# Autodesk Inventor assembly: Intake Assembly
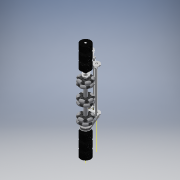
[picture p0: Inventor's stored thumbnail of the model, 180x180]
Saved by Autodesk Inventor 2019.4 (Build 234330000, 330)
## iProperties
Created: 2020-01-28
Part Number: Intake Assembly
Document SubType Name: Assembly
Designer: admin
Mass: 2236.14 g
Surface Area: 6786.27 cm^2
Volume: 1184.94 cm^3
Density: 1.88713 g/cm^3
Author: admin
## Documents named in this file (15)
- C:\Users\admin\Desktop\FRC 2020 Engineering\GitHub\7738-2020\Robot V2\Intake V2\Intake Assembly.iam
- C:\Users\admin\Desktop\FRC 2020 Engineering\GitHub\7738-2020\Robot V2\Intake V2\Intake Arm.ipt
- C:\Users\admin\Desktop\FRC 2020 Engineering\GitHub\7738-2020\Robot V2\Intake V2\Omni Wheel\3_25_Omni-Directional_Wheel_217-4775.iam
- C:\Users\admin\Desktop\FRC 2020 Engineering\GitHub\7738-2020\Robot V2\Turret\775\775pro_775pro_Connect_and_GT2_Pulley_217-6347 (1).iam
- C:\Users\admin\Desktop\FRC 2020 Engineering\GitHub\7738-2020\Robot V2\Intake V2\Intake Assembly\Design Accelerator\Synchronous Belts Transmission1.iam
- C:\Users\admin\Desktop\FRC 2020 Engineering\GitHub\7738-2020\Robot V2\Intake System\MF148ZZ.ipt
- C:\Users\admin\Desktop\FRC 2020 Engineering\GitHub\7738-2020\Robot V2\Turret\F6800.ipt
- C:\Users\admin\Desktop\FRC 2020 Engineering\GitHub\7738-2020\Robot V2\Intake V2\Saftey Axle.ipt
- C:\Users\admin\Desktop\FRC 2020 Engineering\GitHub\7738-2020\Robot V2\Intake V2\Intake Plate Spacer.ipt
- C:\Users\admin\Desktop\FRC 2020 Engineering\GitHub\7738-2020\Robot V2\Intake V2\Intake Axle.ipt
- C:\Users\admin\Desktop\FRC 2020 Engineering\GitHub\7738-2020\Robot V2\Intake V2\Mec Wheel Spacer.ipt
- C:\Users\admin\Desktop\FRC 2020 Engineering\GitHub\7738-2020\Robot V2\Intake V2\Omni Wheel Spacer.ipt
- C:\Users\admin\Desktop\FRC 2020 Engineering\GitHub\7738-2020\Robot V2\Intake V2\Omni Wheel Spacer 2.ipt
- C:\Users\admin\Desktop\FRC 2020 Engineering\GitHub\7738-2020\Robot V2\Intake V2\Pneumatic Spcaer.ipt
- C:\Users\admin\Desktop\FRC 2020 Engineering\GitHub\7738-2020\Robot V2\Intake V2\60mm Mecanum Wheel.ipt
## Components (31 placed, 14 different names)
1. Intake Arm:1 — Mate:1, Mate:2, Mate:3, Mate:4, Mate:5, Mate:6, Mate:7, Mate:9, Mate:10, Mate:11, Mate:13, Mate:15, Mate:18, Mate:23, Mate:60, Mate:61, Mate:65, Mate:66, Mate:68, Mate:84
2. Intake Arm:2 — Mate:1, Mate:2, Mate:3, Mate:8, Mate:16, Mate:17, Mate:21, Mate:22, Mate:55, Mate:56, Mate:57, Mate:58, Mate:59, Mate:62, Mate:82, Mate:91, Mate:92
3. 3_25_Omni-Directional_Wheel_217-4775:1 [sub-assembly] — Mate:4, Mate:86, Mate:88, Mate:89
4. 3_25_Omni-Directional_Wheel_217-4775:2 [sub-assembly] — Mate:5, Mate:90
5. 3_25_Omni-Directional_Wheel_217-4775:3 [sub-assembly] — Mate:6, Mate:85, Mate:87
6. 775pro_775pro_Connect_and_GT2_Pulley_217-6347 (1):1 [sub-assembly] — Mate:9, Mate:10, Mate:23
7. Synchronous Belts Transmission:1 [sub-assembly]
8. MF148ZZ:2 — Mate:11, Mate:13, Mate:53, Mate:54
9. F6800:1 — Mate:15, Mate:18
10. F6800:2 — Mate:16, Mate:17
11. MF148ZZ:4 — Mate:21, Mate:22
12. Saftey Axle:1 — Mate:53, Mate:54
13. Intake Plate Spacer:1 — Mate:55, Mate:57
14. Intake Plate Spacer:2 — Mate:56, Mate:58
15. F6800:3 — Mate:59, Mate:62, Mate:63, Mate:64, Mate:81, Flush:3
16. F6800:4 — Mate:60, Mate:61, Mate:83
17. Intake Axle:1 — Mate:63, Mate:64, Mate:95, Mate:98, Flush:1, Flush:2, Flush:4
18. Mec Wheel Spacer:1 — Mate:65
19. Mec Wheel Spacer:2 — Mate:66
20. Mec Wheel Spacer:4 — Mate:68
21. Omni Wheel Spacer:1 — Mate:81, Mate:82, Mate:85
22. Omni Wheel Spacer:2 — Mate:83, Mate:84, Mate:86
23. Omni Wheel Spacer 2:1 — Mate:87, Mate:90
24. Omni Wheel Spacer 2:2 — Mate:88, Mate:89
25. Pneumatic Spcaer:1 — Mate:91, Mate:92
26. 60mm Mecanum Wheel:1 — Mate:94, Mate:95, Flush:4
27. 60mm Mecanum Wheel:2 — Mate:93, Flush:3, Mate:100
28. 60mm Mecanum Wheel:3 — Mate:93, Mate:94, Mate:100
29. 60mm Mecanum Wheel:4 — Mate:96, Mate:97, Mate:98, Flush:1
30. 60mm Mecanum Wheel:5 — Mate:96, Flush:2, Mate:99
31. 60mm Mecanum Wheel:6 — Mate:97, Mate:99
## Relationships (58: Mate 54, Flush 4)
- Mate:1: Intake Arm:1 ↔ Intake Arm:2
- Mate:2: Intake Arm:1 ↔ Intake Arm:2
- Mate:3 (248.6 mm): Intake Arm:1 ↔ Intake Arm:2
- Mate:4: Intake Arm:1 ↔ 3_25_Omni-Directional_Wheel_217-4775:1
- Mate:5: Intake Arm:1 ↔ 3_25_Omni-Directional_Wheel_217-4775:2
- Mate:6: Intake Arm:1 ↔ 3_25_Omni-Directional_Wheel_217-4775:3
- Mate:7: Intake Arm:1
- Mate:8 (119.3 mm): Intake Arm:2
- Mate:9: Intake Arm:1 ↔ 775pro_775pro_Connect_and_GT2_Pulley_217-6347 (1):1
- Mate:10: Intake Arm:1 ↔ 775pro_775pro_Connect_and_GT2_Pulley_217-6347 (1):1
- Mate:11: Intake Arm:1 ↔ MF148ZZ:2
- Mate:13 (0.2 mm): Intake Arm:1 ↔ MF148ZZ:2
- Mate:15: Intake Arm:1 ↔ F6800:1
- Mate:16: Intake Arm:2 ↔ F6800:2
- Mate:17 (0.2 mm): Intake Arm:2 ↔ F6800:2
- Mate:18 (0.2 mm): Intake Arm:1 ↔ F6800:1
- Mate:21: Intake Arm:2 ↔ MF148ZZ:4
- Mate:22 (0.2 mm): Intake Arm:2 ↔ MF148ZZ:4
- Mate:23: Intake Arm:1 ↔ 775pro_775pro_Connect_and_GT2_Pulley_217-6347 (1):1
- Mate:53: MF148ZZ:2 ↔ Saftey Axle:1
- Mate:54: MF148ZZ:2 ↔ Saftey Axle:1
- Mate:55: Intake Arm:2 ↔ Intake Plate Spacer:1
- Mate:56: Intake Arm:2 ↔ Intake Plate Spacer:2
- Mate:57: Intake Arm:2 ↔ Intake Plate Spacer:1
- Mate:58: Intake Arm:2 ↔ Intake Plate Spacer:2
- Mate:59: Intake Arm:2 ↔ F6800:3
- Mate:60: Intake Arm:1 ↔ F6800:4
- Mate:61 (0.2 mm): Intake Arm:1 ↔ F6800:4
- Mate:62 (0.2 mm): Intake Arm:2 ↔ F6800:3
- Mate:63: F6800:3 ↔ Intake Axle:1
- Mate:64: F6800:3 ↔ Intake Axle:1
- Mate:65: Intake Arm:1 ↔ Mec Wheel Spacer:1
- Mate:66: Intake Arm:1 ↔ Mec Wheel Spacer:2
- Mate:68: Intake Arm:1 ↔ Mec Wheel Spacer:4
- Mate:81: F6800:3 ↔ Omni Wheel Spacer:1
- Mate:82: Intake Arm:2 ↔ Omni Wheel Spacer:1
- Mate:83: F6800:4 ↔ Omni Wheel Spacer:2
- Mate:84: Intake Arm:1 ↔ Omni Wheel Spacer:2
- Mate:85 (0.4 mm): 3_25_Omni-Directional_Wheel_217-4775:3 ↔ Omni Wheel Spacer:1
- Mate:86 (0.4 mm): 3_25_Omni-Directional_Wheel_217-4775:1 ↔ Omni Wheel Spacer:2
- Mate:87: 3_25_Omni-Directional_Wheel_217-4775:3 ↔ Omni Wheel Spacer 2:1
- Mate:88: 3_25_Omni-Directional_Wheel_217-4775:1 ↔ Omni Wheel Spacer 2:2
- Mate:89: 3_25_Omni-Directional_Wheel_217-4775:1 ↔ Omni Wheel Spacer 2:2
- Mate:90: 3_25_Omni-Directional_Wheel_217-4775:2 ↔ Omni Wheel Spacer 2:1
- Mate:91: Intake Arm:2 ↔ Pneumatic Spcaer:1
- Mate:92: Intake Arm:2 ↔ Pneumatic Spcaer:1
- Mate:93: 60mm Mecanum Wheel:2 ↔ 60mm Mecanum Wheel:3
- Mate:94: 60mm Mecanum Wheel:1 ↔ 60mm Mecanum Wheel:3
- Mate:95: Intake Axle:1 ↔ 60mm Mecanum Wheel:1
- Mate:96: 60mm Mecanum Wheel:4 ↔ 60mm Mecanum Wheel:5
- Mate:97: 60mm Mecanum Wheel:4 ↔ 60mm Mecanum Wheel:6
- Mate:98: Intake Axle:1 ↔ 60mm Mecanum Wheel:4
- Flush:1: Intake Axle:1 ↔ 60mm Mecanum Wheel:4
- Flush:2: Intake Axle:1 ↔ 60mm Mecanum Wheel:5
- Mate:99 (1.4 mm): 60mm Mecanum Wheel:5 ↔ 60mm Mecanum Wheel:6
- Flush:3 (25.1 mm): F6800:3 ↔ 60mm Mecanum Wheel:2
- Mate:100 (1.4 mm): 60mm Mecanum Wheel:2 ↔ 60mm Mecanum Wheel:3
- Flush:4: Intake Axle:1 ↔ 60mm Mecanum Wheel:1
